# Autodesk Inventor assembly: IFI_FlyWheelAssembly_Jan23_Wide
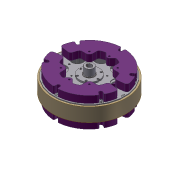
[picture p0: Inventor's stored thumbnail of the model, 180x180]
Saved by Autodesk Inventor 2012 (Build 160160000, 160)
## iProperties
Created: 2012-01-24
Part Number: IFI_FlyWheelAssembly_Jan23_Wide
Document SubType Name: Assembly
Designer: JesseK
Mass: 2197.4 g
Surface Area: 3409.94 cm^2
Volume: 958.094 cm^3
Density: 2.29351 g/cm^3
Translation Standard: STEP AP203
FileName: IFI-WHEEL-ASSY-815-50.STEP
PreProcessor: SolidWorks 2006052
PostProcessor: Build: 160, Release: 2012 RTM - Date: Tue 03/01/2011
Sent Units: inch
Uncertainty: 1e-05
Author: JesseK
## Documents named in this file (8)
- Z:\UserData\Documents\Inventor\team1885frc\Robot2012\Shooter\IFI_FlyWheelAssembly_Jan23_Wide.iam
- Z:\UserData\Documents\Inventor\team1885frc\IFI\Imported Components\IFI-WHEEL-ASSY-815-50\TB-WHEEL-RIM-815 RevG.ipt
- Z:\UserData\Documents\Inventor\team1885frc\IFI\Imported Components\IFI-WHEEL-ASSY-815-50\SBS_SBS0832-0500SS.ipt
- Z:\UserData\Documents\Inventor\team1885frc\IFI\Imported Components\IFI-WHEEL-ASSY-815-50\THF0832-0250-1500.ipt
- Z:\UserData\Documents\Inventor\team1885frc\IFI\Imported Components\IFI-WHEEL-ASSY-815-50\TB-WHEEL-HUB-850 RevG.ipt
- Z:\UserData\Documents\Inventor\team1885frc\IFI\Imported Components\IFI-WHEEL-ASSY-815-50\8x15.ipt
- Z:\UserData\Documents\Inventor\team1885frc\Robot2012\Shooter\IFI_Wheel_Weight_8in.ipt
- Z:\UserData\Documents\Inventor\team1885frc\AndyMark\500EX-Key-Hub.ipt
## Components (30 placed, 7 different names)
1. TB-WHEEL-RIM-815 RevG:1
2. SBS_SBS0832-0500SS:1
3. SBS_SBS0832-0500SS:3
4. THF0832-0250-1500:1
5. SBS_SBS0832-0500SS:4
6. SBS_SBS0832-0500SS:5
7. THF0832-0250-1500:2
8. THF0832-0250-1500:3
9. TB-WHEEL-HUB-850 RevG:1 — Mate:1, Mate:2, Mate:9, Mate:10, Mate:11, Mate:12, Mate:14, Mate:15
10. SBS_SBS0832-0500SS:7
11. SBS_SBS0832-0500SS:8
12. THF0832-0250-1500:4
13. SBS_SBS0832-0500SS:9
14. SBS_SBS0832-0500SS:10
15. SBS_SBS0832-0500SS:11
16. TB-WHEEL-RIM-815 RevG:2
17. SBS_SBS0832-0500SS:12
18. THF0832-0250-1500:5
19. TB-WHEEL-HUB-850 RevG:2 — Mate:3, Mate:4, Mate:5, Mate:6, Mate:7, Mate:8, Mate:13, Mate:16
20. TB-WHEEL-RIM-815 RevG:3
21. SBS_SBS0832-0500SS:13
22. THF0832-0250-1500:6
23. 8x15:1
24. SBS_SBS0832-0500SS:16
25. IFI_Wheel_Weight_8in:1 — Mate:4, Mate:7, Mate:8
26. IFI_Wheel_Weight_8in:2 — Mate:3, Mate:5, Mate:6
27. IFI_Wheel_Weight_8in:3 — Mate:2, Mate:9, Mate:11
28. IFI_Wheel_Weight_8in:4 — Mate:1, Mate:10, Mate:12
29. 500EX-Key-Hub:1 — Mate:13, Mate:16
30. 500EX-Key-Hub:2 — Mate:14, Mate:15
## Relationships (16: Mate 16)
- Mate:1: TB-WHEEL-HUB-850 RevG:1 ↔ IFI_Wheel_Weight_8in:4
- Mate:2: TB-WHEEL-HUB-850 RevG:1 ↔ IFI_Wheel_Weight_8in:3
- Mate:3: TB-WHEEL-HUB-850 RevG:2 ↔ IFI_Wheel_Weight_8in:2
- Mate:4: TB-WHEEL-HUB-850 RevG:2 ↔ IFI_Wheel_Weight_8in:1
- Mate:5: TB-WHEEL-HUB-850 RevG:2 ↔ IFI_Wheel_Weight_8in:2
- Mate:6: TB-WHEEL-HUB-850 RevG:2 ↔ IFI_Wheel_Weight_8in:2
- Mate:7: TB-WHEEL-HUB-850 RevG:2 ↔ IFI_Wheel_Weight_8in:1
- Mate:8: TB-WHEEL-HUB-850 RevG:2 ↔ IFI_Wheel_Weight_8in:1
- Mate:9: TB-WHEEL-HUB-850 RevG:1 ↔ IFI_Wheel_Weight_8in:3
- Mate:10: TB-WHEEL-HUB-850 RevG:1 ↔ IFI_Wheel_Weight_8in:4
- Mate:11: TB-WHEEL-HUB-850 RevG:1 ↔ IFI_Wheel_Weight_8in:3
- Mate:12: TB-WHEEL-HUB-850 RevG:1 ↔ IFI_Wheel_Weight_8in:4
- Mate:13: TB-WHEEL-HUB-850 RevG:2 ↔ 500EX-Key-Hub:1
- Mate:14: TB-WHEEL-HUB-850 RevG:1 ↔ 500EX-Key-Hub:2
- Mate:15: TB-WHEEL-HUB-850 RevG:1 ↔ 500EX-Key-Hub:2
- Mate:16: TB-WHEEL-HUB-850 RevG:2 ↔ 500EX-Key-Hub:1
